# Autodesk Inventor assembly: Spidey
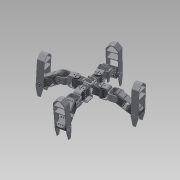
[picture p0: Inventor's stored thumbnail of the model, 180x180]
Saved by Autodesk Inventor 2014 (Build 180170000, 170)
## iProperties
Created: 2014-03-07
Part Number: Spidey
Document SubType Name: Assembly
Designer: Grégoire
Author: Grégoire
## Documents named in this file (9)
- C:\Users\Grégoire\Desktop\XL320\spidey\Spidey.iam
- C:\Users\Grégoire\Desktop\XL320\src\Motor.ipt
- C:\Users\Grégoire\Desktop\XL320\src\Arm.ipt
- C:\Users\Grégoire\Desktop\XL320\src\CounterArm.ipt
- C:\Users\Grégoire\Desktop\XL320\spidey\Ufix.ipt
- C:\Users\Grégoire\Desktop\XL320\spidey\SideToSide.ipt
- C:\Users\Grégoire\Desktop\XL320\spidey\Leg.ipt
- C:\Users\Grégoire\Desktop\XL320\spidey\Body.ipt
- C:\Users\Grégoire\Desktop\XL320\spidey\BodyToOpenCM.ipt
## Components (60 placed, 8 different names)
1. Motor:4 — Placage:132, Placage:133, Placage:135, Placage:148
2. Arm:4
3. CounterArm:4
4. Ufix:3
5. Ufix:4
6. Motor:5
7. Arm:5
8. CounterArm:5
9. SideToSide:3
10. SideToSide:4
11. Motor:6
12. Arm:6
13. CounterArm:6
14. Leg:2
15. Motor:7 — Placage:127, Placage:128, Placage:134, Placage:137, Placage:138
16. Arm:7
17. CounterArm:7
18. Ufix:5
19. Ufix:6
20. Motor:8
21. Arm:8
22. CounterArm:8
23. SideToSide:5
24. SideToSide:6
25. Motor:9
26. Arm:9
27. CounterArm:9
28. Leg:3
29. Motor:10 — Placage:129, Placage:146, Placage:147
30. Arm:10
31. CounterArm:10
32. Ufix:7
33. Ufix:8
34. Motor:11
35. Arm:11
36. CounterArm:11
37. SideToSide:7
38. SideToSide:8
39. Motor:12
40. Arm:12
41. CounterArm:12
42. Leg:4
43. Body:1 — Placage:127, Placage:128, Placage:129, Placage:130, Placage:131, Placage:132, Placage:133, Placage:148
44. Body:2 — Placage:134, Placage:135, Placage:136, Placage:137, Placage:138, Placage:139, Placage:140, Placage:141, Placage:142, Placage:143, Placage:144, Placage:145, Placage:146, Placage:147
45. BodyToOpenCM:1 — Placage:139, Placage:140, Placage:141
46. BodyToOpenCM:2 — Placage:142, Placage:143, Placage:144
47. Ufix:1 — Placage:7, Placage:8, Placage:9, Placage:14, Placage:15
48. Ufix:2 — Placage:5, Placage:6, Placage:7, Placage:8, Placage:9
49. SideToSide:1 — Placage:19, Placage:20, Placage:21, Placage:26, Placage:27, Placage:28
50. SideToSide:2 — Placage:16, Placage:17, Placage:18
51. Leg:1 — Placage:29, Placage:30
52. Motor:1 — Placage:1, Placage:2, Placage:3, Placage:4, Placage:130, Placage:131, Placage:136, Placage:145
53. Arm:1 — Placage:3, Placage:4, Placage:5, Placage:6
54. CounterArm:1 — Placage:1, Placage:2
55. Motor:2 — Placage:16, Placage:17, Placage:18, Placage:19, Placage:20, Placage:21
56. Arm:2 — Placage:15
57. CounterArm:2 — Placage:14
58. Motor:3 — Placage:26, Placage:27, Placage:28
59. Arm:3 — Placage:29, Placage:30
60. CounterArm:3
## Relationships (142: Mate 142)
- Placage:1 [Mate]: Motor:1 ↔ CounterArm:1
- Placage:2 [Mate]: Motor:1 ↔ CounterArm:1
- Placage:3 [Mate]: Motor:1 ↔ Arm:1
- Placage:4 [Mate]: Motor:1 ↔ Arm:1
- Placage:5 [Mate]: Ufix:2 ↔ Arm:1
- Placage:6 [Mate]: Ufix:2 ↔ Arm:1
- Placage:7 [Mate]: Ufix:1 ↔ Ufix:2
- Placage:8 [Mate]: Ufix:1 ↔ Ufix:2
- Placage:9 [Mate]: Ufix:1 ↔ Ufix:2
- [Mate]: Motor:2 ↔ CounterArm:2
- [Mate]: Motor:2 ↔ CounterArm:2
- [Mate]: Motor:2 ↔ Arm:2
- [Mate]: Motor:2 ↔ Arm:2
- Placage:14 [Mate]: Ufix:1 ↔ CounterArm:2
- Placage:15 [Mate]: Ufix:1 ↔ Arm:2
- Placage:16 [Mate]: SideToSide:2 ↔ Motor:2
- Placage:17 [Mate]: SideToSide:2 ↔ Motor:2
- Placage:18 [Mate]: SideToSide:2 ↔ Motor:2
- Placage:19 [Mate]: SideToSide:1 ↔ Motor:2
- Placage:20 [Mate]: SideToSide:1 ↔ Motor:2
- Placage:21 [Mate]: SideToSide:1 ↔ Motor:2
- [Mate]: Motor:3 ↔ CounterArm:3
- [Mate]: Motor:3 ↔ CounterArm:3
- [Mate]: Motor:3 ↔ Arm:3
- [Mate]: Motor:3 ↔ Arm:3
- Placage:26 [Mate]: SideToSide:1 ↔ Motor:3
- Placage:27 [Mate]: SideToSide:1 ↔ Motor:3
- Placage:28 [Mate]: SideToSide:1 ↔ Motor:3
- Placage:29 [Mate]: Leg:1 ↔ Arm:3
- Placage:30 [Mate]: Leg:1 ↔ Arm:3
- [Mate]: Motor:4 ↔ CounterArm:4
- [Mate]: Motor:4 ↔ CounterArm:4
- [Mate]: Motor:4 ↔ Arm:4
- [Mate]: Motor:4 ↔ Arm:4
- [Mate]: Arm:4 ↔ Ufix:4
- [Mate]: Arm:4 ↔ Ufix:4
- [Mate]: Ufix:3 ↔ Ufix:4
- [Mate]: Ufix:3 ↔ Ufix:4
- [Mate]: Ufix:3 ↔ Ufix:4
- [Mate]: Motor:5 ↔ CounterArm:5
- [Mate]: Motor:5 ↔ CounterArm:5
- [Mate]: Motor:5 ↔ Arm:5
- [Mate]: Motor:5 ↔ Arm:5
- [Mate]: Ufix:3 ↔ CounterArm:5
- [Mate]: Ufix:3 ↔ Arm:5
- [Mate]: Motor:5 ↔ SideToSide:4
- [Mate]: Motor:5 ↔ SideToSide:4
- [Mate]: Motor:5 ↔ SideToSide:4
- [Mate]: Motor:5 ↔ SideToSide:3
- [Mate]: Motor:5 ↔ SideToSide:3
- [Mate]: Motor:5 ↔ SideToSide:3
- [Mate]: Motor:6 ↔ CounterArm:6
- [Mate]: Motor:6 ↔ CounterArm:6
- [Mate]: Motor:6 ↔ Arm:6
- [Mate]: Motor:6 ↔ Arm:6
- [Mate]: SideToSide:3 ↔ Motor:6
- [Mate]: SideToSide:3 ↔ Motor:6
- [Mate]: SideToSide:3 ↔ Motor:6
- [Mate]: Arm:6 ↔ Leg:2
- [Mate]: Arm:6 ↔ Leg:2
- [Mate]: Motor:7 ↔ CounterArm:7
- [Mate]: Motor:7 ↔ CounterArm:7
- [Mate]: Motor:7 ↔ Arm:7
- [Mate]: Motor:7 ↔ Arm:7
- [Mate]: Arm:7 ↔ Ufix:6
- [Mate]: Arm:7 ↔ Ufix:6
- [Mate]: Ufix:5 ↔ Ufix:6
- [Mate]: Ufix:5 ↔ Ufix:6
- [Mate]: Ufix:5 ↔ Ufix:6
- [Mate]: Motor:8 ↔ CounterArm:8
- [Mate]: Motor:8 ↔ CounterArm:8
- [Mate]: Motor:8 ↔ Arm:8
- [Mate]: Motor:8 ↔ Arm:8
- [Mate]: Ufix:5 ↔ CounterArm:8
- [Mate]: Ufix:5 ↔ Arm:8
- [Mate]: Motor:8 ↔ SideToSide:6
- [Mate]: Motor:8 ↔ SideToSide:6
- [Mate]: Motor:8 ↔ SideToSide:6
- [Mate]: Motor:8 ↔ SideToSide:5
- [Mate]: Motor:8 ↔ SideToSide:5
- [Mate]: Motor:8 ↔ SideToSide:5
- [Mate]: Motor:9 ↔ CounterArm:9
- [Mate]: Motor:9 ↔ CounterArm:9
- [Mate]: Motor:9 ↔ Arm:9
- [Mate]: Motor:9 ↔ Arm:9
- [Mate]: SideToSide:5 ↔ Motor:9
- [Mate]: SideToSide:5 ↔ Motor:9
- [Mate]: SideToSide:5 ↔ Motor:9
- [Mate]: Arm:9 ↔ Leg:3
- [Mate]: Arm:9 ↔ Leg:3
- [Mate]: Motor:10 ↔ CounterArm:10
- [Mate]: Motor:10 ↔ CounterArm:10
- [Mate]: Motor:10 ↔ Arm:10
- [Mate]: Motor:10 ↔ Arm:10
- [Mate]: Arm:10 ↔ Ufix:8
- [Mate]: Arm:10 ↔ Ufix:8
- [Mate]: Ufix:7 ↔ Ufix:8
- [Mate]: Ufix:7 ↔ Ufix:8
- [Mate]: Ufix:7 ↔ Ufix:8
- [Mate]: Motor:11 ↔ CounterArm:11
- [Mate]: Motor:11 ↔ CounterArm:11
- [Mate]: Motor:11 ↔ Arm:11
- [Mate]: Motor:11 ↔ Arm:11
- [Mate]: Ufix:7 ↔ CounterArm:11
- [Mate]: Ufix:7 ↔ Arm:11
- [Mate]: Motor:11 ↔ SideToSide:8
- [Mate]: Motor:11 ↔ SideToSide:8
- [Mate]: Motor:11 ↔ SideToSide:8
- [Mate]: Motor:11 ↔ SideToSide:7
- [Mate]: Motor:11 ↔ SideToSide:7
- [Mate]: Motor:11 ↔ SideToSide:7
- [Mate]: Motor:12 ↔ CounterArm:12
- [Mate]: Motor:12 ↔ CounterArm:12
- [Mate]: Motor:12 ↔ Arm:12
- [Mate]: Motor:12 ↔ Arm:12
- [Mate]: SideToSide:7 ↔ Motor:12
- [Mate]: SideToSide:7 ↔ Motor:12
- [Mate]: SideToSide:7 ↔ Motor:12
- [Mate]: Arm:12 ↔ Leg:4
- [Mate]: Arm:12 ↔ Leg:4
- Placage:127 [Mate]: Motor:7 ↔ Body:1
- Placage:128 [Mate]: Motor:7 ↔ Body:1
- Placage:129 [Mate]: Motor:10 ↔ Body:1
- Placage:130 [Mate]: Body:1 ↔ Motor:1
- Placage:131 [Mate]: Body:1 ↔ Motor:1
- Placage:132 [Mate]: Motor:4 ↔ Body:1
- Placage:133 [Mate]: Motor:4 ↔ Body:1
- Placage:134 [Mate]: Motor:7 ↔ Body:2
- Placage:135 [Mate]: Motor:4 ↔ Body:2
- Placage:136 [Mate]: Body:2 ↔ Motor:1
- Placage:137 [Mate]: Motor:7 ↔ Body:2
- Placage:138 [Mate]: Motor:7 ↔ Body:2
- Placage:139 [Mate]: Body:2 ↔ BodyToOpenCM:1
- Placage:140 [Mate]: Body:2 ↔ BodyToOpenCM:1
- Placage:141 [Mate]: Body:2 ↔ BodyToOpenCM:1
- Placage:142 [Mate]: Body:2 ↔ BodyToOpenCM:2
- Placage:143 [Mate]: Body:2 ↔ BodyToOpenCM:2
- Placage:144 [Mate]: Body:2 ↔ BodyToOpenCM:2
- Placage:145 [Mate]: Body:2 ↔ Motor:1
- Placage:146 [Mate]: Motor:10 ↔ Body:2
- Placage:147 [Mate]: Motor:10 ↔ Body:2
- Placage:148 [Mate]: Motor:4 ↔ Body:1
## Named parameters: d25_d0 = 0 mm, d26_d1 = 0 mm, d27_d2 = 0 mm, d28_d3 = 0 mm, d37_d0 = 0 mm, d38_d1 = 0 mm, d39_d2 = 0 mm, d40_d3 = 0 mm, d52_d0 = 0 mm, d53_d1 = 0 mm, d54_d2 = 0 mm, d55_d3 = 0 mm, d56_d20 = 0 mm, d57_d21 = 0 mm, d58_d22 = 0 mm, d59_d23 = 0 mm, d60_d24 = 0 mm, d61_d25_d0 = 0 mm, d62_d26_d1 = 0 mm, d63_d27_d2 = 0 mm, d64_d28_d3 = 0 mm, d65_d29 = 0 mm, d66_d30 = 0 mm, d67_d31 = 0 mm, d68_d32 = 0 mm, d69_d33 = 0 mm, d70_d34 = 0 mm, d71_d35 = 0 mm, d72_d36 = 0 mm, d73_d37_d0 = 0 mm, d74_d38_d1 = 0 mm, d75_d39_d2 = 0 mm, d76_d40_d3 = 0 mm, d77_d41 = 0 mm, d78_d42 = 0 mm, d79_d43 = 0 mm, d80_d44 = 0 mm, d81_d45 = 0 mm, d82_d0 = 0 mm, d83_d1 = 0 mm, d84_d2 = 0 mm, d85_d3 = 0 mm, d86_d20 = 0 mm, d87_d21 = 0 mm, d88_d22 = 0 mm, d89_d23 = 0 mm, d90_d24 = 0 mm, d91_d25_d0 = 0 mm, d92_d26_d1 = 0 mm, d93_d27_d2 = 0 mm, d94_d28_d3 = 0 mm, d95_d29 = 0 mm, d96_d30 = 0 mm, d97_d31 = 0 mm, d98_d32 = 0 mm, d99_d33 = 0 mm, d100_d34 = 0 mm, d101_d35 = 0 mm, d102_d36 = 0 mm, d103_d37_d0 = 0 mm, d104_d38_d1 = 0 mm, d105_d39_d2 = 0 mm, d106_d40_d3 = 0 mm, d107_d41 = 0 mm, d108_d42 = 0 mm, d109_d43 = 0 mm, d110_d44 = 0 mm, d111_d45 = 0 mm, d112_d0 = 0 mm, d113_d1 = 0 mm, d114_d2 = 0 mm, d115_d3 = 0 mm, d116_d20 = 0 mm, d117_d21 = 0 mm, d118_d22 = 0 mm, d119_d23 = 0 mm, d120_d24 = 0 mm, d121_d25_d0 = 0 mm, d122_d26_d1 = 0 mm, d123_d27_d2 = 0 mm, d124_d28_d3 = 0 mm, d125_d29 = 0 mm, d126_d30 = 0 mm, d127_d31 = 0 mm, d128_d32 = 0 mm, d129_d33 = 0 mm, d130_d34 = 0 mm, d131_d35 = 0 mm, d132_d36 = 0 mm, d133_d37_d0 = 0 mm, d134_d38_d1 = 0 mm, d135_d39_d2 = 0 mm, d136_d40_d3 = 0 mm, d137_d41 = 0 mm, d138_d42 = 0 mm, d139_d43 = 0 mm, d140_d44 = 0 mm, d141_d45 = 0 mm
